# Autodesk Inventor assembly: Tracks Drag Chain Assembly_MIR
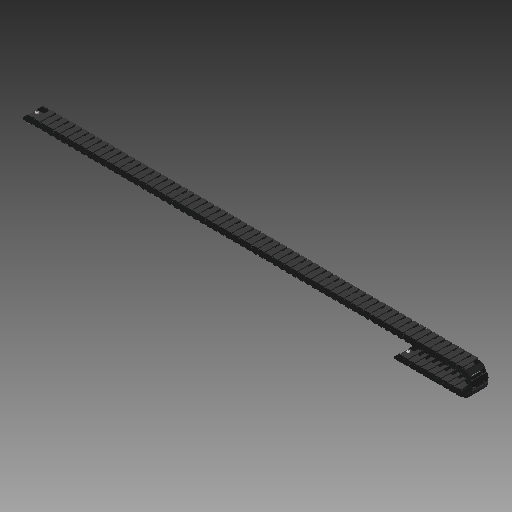
[picture p0: Inventor's stored thumbnail of the model, 512x512]
Saved by Autodesk Inventor 2017 (Build 210142000, 142)
## iProperties
Created: 2014-07-23
Part Number: Tracks Drag Chain Assembly_MIR
Document SubType Name: Assembly
Designer: Ali
Author: umr
Sending System: SolidWorks 2014
Last Author: Rory
Last Saved: 2016-05-10
## Documents named in this file (7)
- C:\Users\Ali\Desktop\roboticFarm-master\Models2\CableCarier\Tracks Drag Chain Assembly_MIR.iam
- C:\Users\Ali\Desktop\roboticFarm-master\Original\SolidWorks 2014 Files\Drag Chain Link_MIR.ipt
- C:\Users\Ali\Desktop\roboticFarm-master\Original\SolidWorks 2014 Files\Drag Chain End 1_MIR.ipt
- C:\Users\Ali\Desktop\roboticFarm-master\Original\SolidWorks 2014 Files\Drag Chain End 2_MIR.ipt
- C:\Users\Ali\Desktop\roboticFarm-master\Models2\CableCarier\M5 Locknut_MIR.ipt
- C:\Users\Ali\Desktop\roboticFarm-master\Models2\CableCarier\M5 Screw_16mm_MIR.ipt
- C:\Users\Ali\Desktop\roboticFarm-master\Models2\CableCarier\M5 Washer_MIR.ipt
## Components (92 placed, 6 different names)
1. Drag Chain Link_MIR:1
2. Drag Chain Link_MIR:2
3. Drag Chain Link_MIR:3
4. Drag Chain Link_MIR:4
5. Drag Chain Link_MIR:5
6. Drag Chain Link_MIR:6
7. Drag Chain Link_MIR:7
8. Drag Chain Link_MIR:8
9. Drag Chain Link_MIR:9
10. Drag Chain Link_MIR:10
11. Drag Chain Link_MIR:11
12. Drag Chain Link_MIR:12
13. Drag Chain Link_MIR:13
14. Drag Chain Link_MIR:14
15. Drag Chain Link_MIR:15
16. Drag Chain Link_MIR:16
17. Drag Chain Link_MIR:17
18. Drag Chain Link_MIR:18
19. Drag Chain Link_MIR:19
20. Drag Chain Link_MIR:20
21. Drag Chain Link_MIR:21
22. Drag Chain Link_MIR:22
23. Drag Chain Link_MIR:23
24. Drag Chain Link_MIR:24
25. Drag Chain Link_MIR:25
26. Drag Chain Link_MIR:26
27. Drag Chain Link_MIR:27
28. Drag Chain Link_MIR:28
29. Drag Chain Link_MIR:29
30. Drag Chain Link_MIR:30
31. Drag Chain Link_MIR:31
32. Drag Chain Link_MIR:32
33. Drag Chain Link_MIR:33
34. Drag Chain Link_MIR:34
35. Drag Chain Link_MIR:35
36. Drag Chain Link_MIR:36
37. Drag Chain Link_MIR:37
38. Drag Chain Link_MIR:38
39. Drag Chain Link_MIR:39
40. Drag Chain Link_MIR:40
41. Drag Chain Link_MIR:41
42. Drag Chain Link_MIR:42
43. Drag Chain Link_MIR:43
44. Drag Chain Link_MIR:44
45. Drag Chain Link_MIR:45
46. Drag Chain Link_MIR:46
47. Drag Chain Link_MIR:47
48. Drag Chain Link_MIR:48
49. Drag Chain Link_MIR:49
50. Drag Chain Link_MIR:50
51. Drag Chain Link_MIR:51
52. Drag Chain Link_MIR:52
53. Drag Chain Link_MIR:53
54. Drag Chain Link_MIR:54
55. Drag Chain Link_MIR:55
56. Drag Chain Link_MIR:56
57. Drag Chain Link_MIR:57
58. Drag Chain Link_MIR:58
59. Drag Chain Link_MIR:59
60. Drag Chain Link_MIR:60
61. Drag Chain Link_MIR:61
62. Drag Chain Link_MIR:62
63. Drag Chain End 1_MIR:1 — Rigid:15, Rigid:16, Rigid:13, Rigid:14
64. Drag Chain End 2_MIR:1 — Rigid:11, Rigid:9, Rigid:10, Rigid:12
65. Drag Chain Link_MIR:63
66. Drag Chain Link_MIR:64
67. Drag Chain Link_MIR:65
68. Drag Chain Link_MIR:66
69. Drag Chain Link_MIR:67
70. Drag Chain Link_MIR:68
71. Drag Chain Link_MIR:69
72. Drag Chain Link_MIR:70
73. Drag Chain Link_MIR:71
74. Drag Chain Link_MIR:72
75. Drag Chain Link_MIR:73
76. Drag Chain Link_MIR:74
77. Drag Chain Link_MIR:75
78. Drag Chain Link_MIR:76
79. Drag Chain Link_MIR:77
80. Drag Chain Link_MIR:78
81. M5 Locknut_MIR:1 — Rigid:2
82. M5 Screw_16mm_MIR:1 — Rigid:15
83. M5 Washer_MIR:1 — Rigid:16, Rigid:2
84. M5 Locknut_MIR:2 — Rigid:7
85. M5 Screw_16mm_MIR:2 — Rigid:13
86. M5 Locknut_MIR:3 — Rigid:8
87. M5 Screw_16mm_MIR:3 — Rigid:11
88. M5 Locknut_MIR:4 — Rigid:6
89. M5 Screw_16mm_MIR:4 — Rigid:9
90. M5 Washer_MIR:2 — Rigid:10, Rigid:7
91. M5 Washer_MIR:3 — Rigid:12, Rigid:6
92. M5 Washer_MIR:4 — Rigid:14, Rigid:8
## Relationships (12: WeldJoint 12)
- Rigid:15 [WeldJoint]: Drag Chain End 1_MIR:1 ↔ M5 Screw_16mm_MIR:1
- Rigid:16 [WeldJoint]: Drag Chain End 1_MIR:1 ↔ M5 Washer_MIR:1
- Rigid:2 [WeldJoint]: M5 Locknut_MIR:1 ↔ M5 Washer_MIR:1
- Rigid:13 [WeldJoint]: Drag Chain End 1_MIR:1 ↔ M5 Screw_16mm_MIR:2
- Rigid:11 [WeldJoint]: Drag Chain End 2_MIR:1 ↔ M5 Screw_16mm_MIR:3
- Rigid:9 [WeldJoint]: Drag Chain End 2_MIR:1 ↔ M5 Screw_16mm_MIR:4
- Rigid:10 [WeldJoint]: Drag Chain End 2_MIR:1 ↔ M5 Washer_MIR:2
- Rigid:7 [WeldJoint]: M5 Locknut_MIR:2 ↔ M5 Washer_MIR:2
- Rigid:12 [WeldJoint]: Drag Chain End 2_MIR:1 ↔ M5 Washer_MIR:3
- Rigid:6 [WeldJoint]: M5 Locknut_MIR:4 ↔ M5 Washer_MIR:3
- Rigid:14 [WeldJoint]: Drag Chain End 1_MIR:1 ↔ M5 Washer_MIR:4
- Rigid:8 [WeldJoint]: M5 Locknut_MIR:3 ↔ M5 Washer_MIR:4
